# Autodesk Inventor assembly: all_assembled
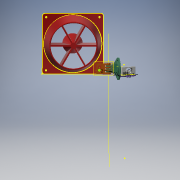
[picture p0: Inventor's stored thumbnail of the model, 180x180]
Saved by Autodesk Inventor 2019 (Build 230136000, 136)
## iProperties
Created: 2020-07-20
Part Number: all_assembled
Document SubType Name: Assembly
Designer: assman
Author: assman
## Documents named in this file (5)
- D:\Inventor\Projects\FanSupport\all_assembled.iam
- D:\Inventor\Projects\FanSupport\plate1.ipt
- D:\Inventor\Projects\FanSupport\mount1.ipt
- D:\Inventor\Projects\FanSupport\mounttest.ipt
- D:\Inventor\Projects\FanSupport\cover.ipt
## Components (4 placed, 4 different names)
1. plate1:1 — Rotational:1
2. mount1:1 — Rotational:1, Rotational:2
3. mounttest:1 — Rotational:2, Rotational:3, Flush:1
4. cover:1 — Rotational:3
## Relationships (4: RevoluteJoint 3, Flush 1)
- Rotational:1 [RevoluteJoint]: plate1:1 ↔ mount1:1
- Rotational:2 [RevoluteJoint] (2.6 mm): mount1:1 ↔ mounttest:1
- Rotational:3 [RevoluteJoint]: mounttest:1 ↔ cover:1
- Flush:1: mounttest:1
